# Autodesk Inventor assembly: правый привод_MIR
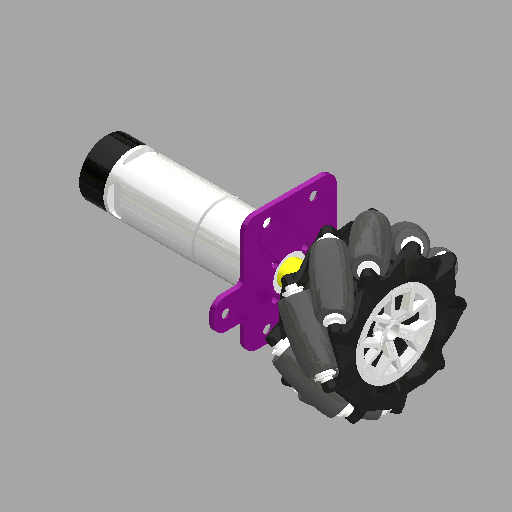
[picture p0: Inventor's stored thumbnail of the model, 512x512]
Saved by Autodesk Inventor 2025 (Build 290162000, 162)
## iProperties
Created: 2025-02-16
Part Number: правый привод_MIR
Document SubType Name: Assembly
Designer: volko
Author: volko
## Documents named in this file (5)
- C:\Users\Artem Sannikov\Desktop\diplom\Модели\детали\правый привод_MIR.iam
- C:\Users\Artem Sannikov\Desktop\diplom\Модели\Mecanum wheel - right\Mecanum wheel - right_MIR.iam
- C:\Users\Artem Sannikov\Desktop\diplom\Модели\детали\CHP-42GP-775 ABHL_MIR1.ipt
- C:\Users\Artem Sannikov\Desktop\diplom\Модели\детали\переходная втулка_MIR1.ipt
- C:\Users\Artem Sannikov\Desktop\diplom\Модели\детали\кронштейн_zerkalo.ipt
## Components (4 placed, 4 different names)
1. Mecanum wheel - right_MIR:1 [sub-assembly] — Совмещение:10, Совмещение:9, Совмещение:8
2. CHP-42GP-775 ABHL_MIR1:1 — Заподлицо:1, Совмещение:2, Совмещение:1, Совмещение:7, Совмещение:6, Совмещение:12
3. переходная втулка_MIR1:1 — Совмещение:10, Совмещение:9, Совмещение:8, Совмещение:7, Совмещение:6, Совмещение:11
4. кронштейн_zerkalo:1 — Совмещение:11, Совмещение:12
## Relationships (10: Mate 9, Flush 1)
- Заподлицо:1 [Flush]: CHP-42GP-775 ABHL_MIR1:1
- Совмещение:2 [Mate]: CHP-42GP-775 ABHL_MIR1:1
- Совмещение:1 [Mate]: CHP-42GP-775 ABHL_MIR1:1
- Совмещение:10 [Mate]: Mecanum wheel - right_MIR:1 ↔ переходная втулка_MIR1:1
- Совмещение:9 [Mate]: Mecanum wheel - right_MIR:1 ↔ переходная втулка_MIR1:1
- Совмещение:8 [Mate]: Mecanum wheel - right_MIR:1 ↔ переходная втулка_MIR1:1
- Совмещение:7 [Mate]: CHP-42GP-775 ABHL_MIR1:1 ↔ переходная втулка_MIR1:1
- Совмещение:6 [Mate]: CHP-42GP-775 ABHL_MIR1:1 ↔ переходная втулка_MIR1:1
- Совмещение:11 [Mate]: переходная втулка_MIR1:1 ↔ кронштейн_zerkalo:1
- Совмещение:12 [Mate]: CHP-42GP-775 ABHL_MIR1:1 ↔ кронштейн_zerkalo:1
